# Autodesk Inventor assembly: SACMI PH1500
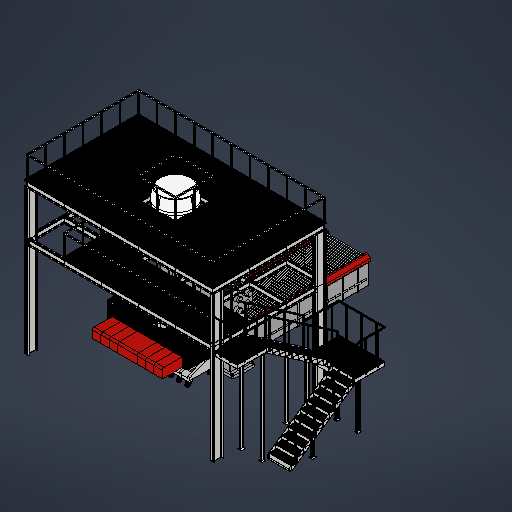
[picture p0: Inventor's stored thumbnail of the model, 512x512]
Saved by Autodesk Inventor 2025 (Build 290162000, 162)
## iProperties
Created: 2024-05-02
Part Number: SACMI PH1500
Document SubType Name: Assembly
Designer: zulet
Author: zulet
## Documents named in this file (18)
- D:\UNAL\2024-1S\APM\Digital Factory\Ceramic Press\SACMI PH1500.iam
- D:\UNAL\2024-1S\APM\Digital Factory\Ceramic Press\SACMI PH1500 30X60 DIE SET BASE.ipt
- D:\UNAL\2024-1S\APM\Digital Factory\Ceramic Press\SACMI PH1500 BASE.ipt
- D:\UNAL\2024-1S\APM\Digital Factory\Ceramic Press\SACMI PH1500 30X60 DIE SET TILES BOTTOM MOLD.ipt
- D:\UNAL\2024-1S\APM\Digital Factory\Ceramic Press\SACMI PH1500 PRESS TOP.ipt
- D:\UNAL\2024-1S\APM\Digital Factory\Ceramic Press\SACMI PH1500 30X60 DIE SET TOP.ipt
- D:\UNAL\2024-1S\APM\Digital Factory\Ceramic Press\SACMI PH1500 POWER FEED SYSTEM.ipt
- D:\UNAL\2024-1S\APM\Digital Factory\Ceramic Press\SACMI PH1500 FILLER BOX GRID-DRIVING.ipt
- D:\UNAL\2024-1S\APM\Digital Factory\Ceramic Press\SACMI PH1500 HOPPER FEEDER.ipt
- D:\UNAL\2024-1S\APM\Digital Factory\Ceramic Press\SACMI PH1500 FEEDER STRUCTURE.ipt
- D:\UNAL\2024-1S\APM\Digital Factory\Ceramic Press\SACMI PH1500\Frame\SACMI PH1500 FEEDER FRAME.iam
- D:\UNAL\2024-1S\APM\Digital Factory\Ceramic Press\platform\StairsFirst.ipt
- D:\UNAL\2024-1S\APM\Digital Factory\Ceramic Press\platform\StairsSecond.ipt
- D:\UNAL\2024-1S\APM\Digital Factory\Ceramic Press\SACMI PH1500 HOPPER.ipt
- D:\UNAL\2024-1S\APM\Digital Factory\Ceramic Press\SACMI PH1500 HOPPER END TUBE.ipt
- D:\UNAL\2024-1S\APM\Digital Factory\Conveyor System\CONVEYOR\CONVEYOR-1500x5000x1140.iam
- D:\UNAL\2024-1S\APM\Digital Factory\Conveyor System\CONVEYOR.iam
- D:\UNAL\2024-1S\APM\Digital Factory\TILE 30X60.ipt
## Components (22 placed, 16 different names)
1. SACMI PH1500 30X60 DIE SET BASE:1 — Mate:1, Flush:1, Flush:2, Slider:1, Rigid:2, Mate:6, Rigid:4
2. SACMI PH1500 BASE:1 — Mate:1, Flush:1, Flush:2, Cylindrical:1, Cylindrical:2, Flush:3, Mate:3, Flush:6, Flush:7
3. SACMI PH1500 30X60 DIE SET TILES BOTTOM MOLD:1 — Slider:1
4. SACMI PH1500 PRESS TOP:1 — Cylindrical:1, Cylindrical:2, Rigid:1
5. SACMI PH1500 30X60 DIE SET TOP:1 — Rigid:1
6. SACMI PH1500 FILLER BOX GRID-DRIVING:1 — Slider:2
7. SACMI PH1500 HOPPER FEEDER:1 — Slider:3, Slider:4
8. SACMI PH1500 FEEDER STRUCTURE:1 — Flush:3, Mate:3, Flush:6, Mate:4
9. SACMI PH1500 FEEDER FRAME:1 [sub-assembly] — Flush:4, Flush:5, Mate:2, Mate:5
10. StairsFirst:1 — Rigid:3
11. StairsSecond:1 — Rigid:3, Flush:4, Flush:5, Mate:2
12. SACMI PH1500 HOPPER:1 — Mate:4, Mate:5
13. SACMI PH1500 HOPPER END TUBE:1 — Slider:4
14. CONVEYOR-1500x5000x1140:1 [sub-assembly] — Mate:6, Flush:7
15. SACMI PH1500 POWER FEED SYSTEM:1 — Rigid:2, Slider:2, Slider:3
16. TILE 30X60:1 — Rigid:4
17. SACMI PH1500 POWER FEED SYSTEM:2
18. TILE 30X60:2
19. SACMI PH1500 POWER FEED SYSTEM:3
20. TILE 30X60:3
21. SACMI PH1500 POWER FEED SYSTEM:4
22. TILE 30X60:4
## Component patterns: (4 elements, first: SACMI PH1500 POWER FEED SYSTEM:1 + TILE 30X60:1)
## Relationships (23: Flush 7, Mate 6, TranslationJoint 4, WeldJoint 4, CylindricalJoint 2)
- Mate:1: SACMI PH1500 30X60 DIE SET BASE:1 ↔ SACMI PH1500 BASE:1
- Flush:1: SACMI PH1500 30X60 DIE SET BASE:1 ↔ SACMI PH1500 BASE:1
- Flush:2: SACMI PH1500 30X60 DIE SET BASE:1 ↔ SACMI PH1500 BASE:1
- Slider:1 [TranslationJoint]: SACMI PH1500 30X60 DIE SET BASE:1 ↔ SACMI PH1500 30X60 DIE SET TILES BOTTOM MOLD:1
- Cylindrical:1: SACMI PH1500 BASE:1 ↔ SACMI PH1500 PRESS TOP:1
- Cylindrical:2: SACMI PH1500 BASE:1 ↔ SACMI PH1500 PRESS TOP:1
- Rigid:1 [WeldJoint]: SACMI PH1500 PRESS TOP:1 ↔ SACMI PH1500 30X60 DIE SET TOP:1
- Rigid:2 [WeldJoint]: SACMI PH1500 30X60 DIE SET BASE:1 ↔ SACMI PH1500 POWER FEED SYSTEM:1
- Slider:2 [TranslationJoint]: SACMI PH1500 FILLER BOX GRID-DRIVING:1 ↔ SACMI PH1500 POWER FEED SYSTEM:1
- Slider:3 [TranslationJoint]: SACMI PH1500 HOPPER FEEDER:1 ↔ SACMI PH1500 POWER FEED SYSTEM:1
- Flush:3: SACMI PH1500 BASE:1 ↔ SACMI PH1500 FEEDER STRUCTURE:1
- Rigid:3 [WeldJoint]: StairsFirst:1 ↔ StairsSecond:1
- Flush:4: SACMI PH1500 FEEDER FRAME:1 ↔ StairsSecond:1
- Flush:5: SACMI PH1500 FEEDER FRAME:1 ↔ StairsSecond:1
- Mate:2: SACMI PH1500 FEEDER FRAME:1 ↔ StairsSecond:1
- Mate:3 (-1500 mm): SACMI PH1500 BASE:1 ↔ SACMI PH1500 FEEDER STRUCTURE:1
- Flush:6: SACMI PH1500 BASE:1 ↔ SACMI PH1500 FEEDER STRUCTURE:1
- Mate:4: SACMI PH1500 FEEDER STRUCTURE:1 ↔ SACMI PH1500 HOPPER:1
- Mate:5: SACMI PH1500 FEEDER FRAME:1 ↔ SACMI PH1500 HOPPER:1
- Slider:4 [TranslationJoint]: SACMI PH1500 HOPPER FEEDER:1 ↔ SACMI PH1500 HOPPER END TUBE:1
- Mate:6: SACMI PH1500 30X60 DIE SET BASE:1 ↔ CONVEYOR-1500x5000x1140:1
- Flush:7: SACMI PH1500 BASE:1 ↔ CONVEYOR-1500x5000x1140:1
- Rigid:4 [WeldJoint]: SACMI PH1500 30X60 DIE SET BASE:1 ↔ TILE 30X60:1
